# Autodesk Inventor assembly: mizuno-pipe
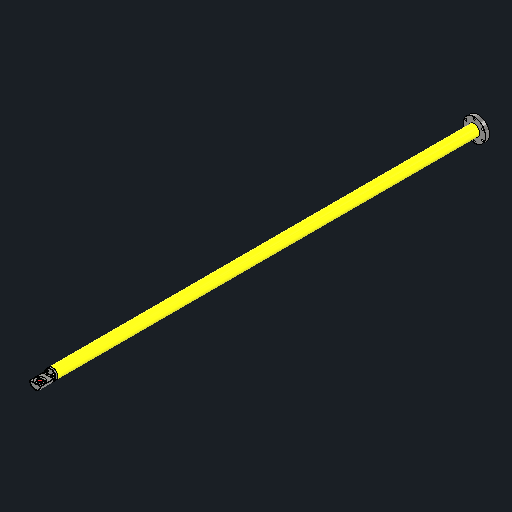
[picture p0: Inventor's stored thumbnail of the model, 512x512]
Saved by Autodesk Inventor 2027.1 (Build 311270010, 270A)
## iProperties
Created: 2026-05-08
Part Number: mizuno-pipe
Document SubType Name: Assembly
Designer: zetsu
Author: zetsu
## Documents named in this file (4)
- C:\Users\queezz\Dropbox\Drawings\pihti-cad\bellows-probe\mizuno-pipe.iam
- C:\Users\queezz\Dropbox\Drawings\pihti-cad\bellows-probe\mizuno-probe-head.iam
- C:\Users\queezz\Dropbox\Drawings\pihti-cad\bellows-probe\pipe-for-mizuno-probe.ipt
- C:\Users\queezz\Dropbox\Drawings\pihti-cad\PALP\Prototype-PALP-CF70-34-hole-flange.ipt
## Components (3 placed, 3 different names)
1. mizuno-probe-head:1 [sub-assembly] — Rigid:1
2. pipe-for-mizuno-probe:1 — Rigid:1, CF70 weld flange to pipe end - rigid
3. CF70 weld flange for 34 mm pipe:1 — CF70 weld flange to pipe end - rigid
## Relationships (2: WeldJoint 2)
- Rigid:1 [WeldJoint]: mizuno-probe-head:1 ↔ pipe-for-mizuno-probe:1
- CF70 weld flange to pipe end - rigid [WeldJoint]: pipe-for-mizuno-probe:1 ↔ CF70 weld flange for 34 mm pipe:1
